# Autodesk Inventor assembly: robot_frame_layer1
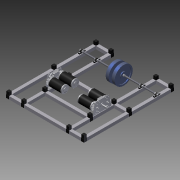
[picture p0: Inventor's stored thumbnail of the model, 180x180]
Saved by Autodesk Inventor 2011 (Build 150239000, 239)
## iProperties
Created: 2013-01-17
Part Number: robot_frame_layer1
Document SubType Name: Assembly
Designer: Christopher
Author: Christopher
## Documents named in this file (19)
- F:\Users\Christopher\Documents\GitHub\2013CAD\2013 robot\forklift\robot parts\robot_frame_layer1.iam
- F:\Users\Christopher\Documents\GitHub\2013CAD\2013 robot\forklift\robot parts\1tube_4_layer1_outside.ipt
- F:\Users\Christopher\Documents\GitHub\2013CAD\2013 robot\forklift\robot parts\1tube_6_layer1_boardsupportsupport.ipt
- F:\Users\Christopher\Documents\GitHub\2013CAD\2013 robot\forklift\robot parts\1tube_6_layer1_motorsupport.ipt
- F:\Users\Christopher\Documents\GitHub\2013CAD\2013 robot\forklift\robot parts\1tube_14_layer1_innersupport.ipt
- F:\Users\Christopher\Documents\GitHub\2013CAD\2013 robot\forklift\robot parts\1tube_14_layer1_inside.ipt
- F:\Users\Christopher\Documents\GitHub\2013CAD\2013 robot\forklift\robot parts\1tube_14_layer1_outside.ipt
- F:\Users\Christopher\Documents\GitHub\2013CAD\2013 robot\forklift\Misc parts\3-way corner.ipt
- F:\Users\Christopher\Documents\GitHub\2013CAD\2013 robot\forklift\Misc parts\4-way corner.ipt
- F:\Users\Christopher\Documents\GitHub\2013CAD\2013 robot\forklift\Misc parts\5-way corner.ipt
- F:\Users\Christopher\Documents\GitHub\2013CAD\2013 robot\forklift\robot parts\1tube_13_layer1_side.ipt
- F:\Users\Christopher\Documents\GitHub\2013CAD\2013 robot\forklift\Chassis\Chassis_CIMGearbox_AndyMark_am-0734.ipt
- F:\Users\Christopher\Documents\GitHub\2013CAD\2013 robot\forklift\Misc parts\.5inch_side_bearing.ipt
- F:\Users\Christopher\Documents\GitHub\2013CAD\2013 robot\forklift\Misc parts\1.5_bolt_.25_20.ipt
- F:\Users\Christopher\Documents\GitHub\2013CAD\2013 robot\forklift\Misc parts\nut_.25_20.ipt
- F:\Users\Christopher\Documents\GitHub\2013CAD\2013 robot\forklift\Misc parts\.5_inch_axle_bushing.ipt
- F:\Users\Christopher\Documents\GitHub\2013CAD\2013 robot\forklift\robot parts\example_wheel_6inch_.5axle.ipt
- F:\Users\Christopher\Documents\GitHub\2013CAD\2013 robot\forklift\frame parts\0.5unkeyedaxle_26.ipt
- F:\Users\Christopher\Documents\GitHub\2013CAD\2013 robot\forklift\frame parts\corner_prop.ipt
## Components (70 placed, 18 different names)
1. 1tube_4_layer1_outside:1 — Mate:7, Mate:8, Mate:9, Mate:10, Mate:11, Mate:12
2. 1tube_6_layer1_boardsupportsupport:1 — Mate:22, Mate:23, Mate:24, Mate:25, Mate:26, Mate:27
3. 1tube_6_layer1_motorsupport:1 — Mate:28, Mate:29, Mate:30, Mate:110, Flush:1, Mate:120, Flush:2
4. 1tube_14_layer1_innersupport:1 — Mate:31, Mate:32, Mate:33, Mate:46, Mate:47, Mate:48
5. 1tube_14_layer1_outside:1 — Mate:19, Mate:20, Mate:21, Mate:49, Mate:50, Mate:51
6. 3-way corner:1 — Mate:13, Mate:14, Mate:15, Mate:150, Mate:151
7. 3-way corner:2 — Mate:7, Mate:8, Mate:9, Mate:148
8. 3-way corner:4 — Mate:70, Mate:71, Mate:72, Mate:121, Mate:122, Mate:131
9. 3-way corner:5 — Mate:73, Mate:74, Mate:75, Mate:152, Flush:12, Flush:13, Mate:153
10. 3-way corner:6 — Mate:67, Mate:68, Mate:69, Flush:8, Flush:9
11. 3-way corner:7 — Mate:16, Mate:17, Mate:18, Mate:142, Mate:143, Mate:144
12. 4-way corner:2 — Mate:10, Mate:11, Mate:12, Mate:19, Mate:20, Mate:21, Mate:22, Mate:23, Mate:24
13. 1tube_4_layer1_outside:2 — Mate:13, Mate:14, Mate:15, Mate:16, Mate:17, Mate:18
14. 4-way corner:3 — Mate:25, Mate:26, Mate:27, Mate:28, Mate:29, Mate:30, Mate:31, Mate:32, Mate:33
15. 1tube_14_layer1_innersupport:2 — Mate:82, Mate:83, Mate:91, Mate:101, Mate:102, Mate:103
16. 4-way corner:5 — Mate:46, Mate:47, Mate:48, Mate:53, Mate:54, Mate:128, Mate:129, Mate:130
17. 4-way corner:6 — Mate:49, Mate:50, Mate:51, Mate:52, Mate:64, Mate:65, Mate:66
18. 1tube_6_layer1_motorsupport:2 — Mate:127, Flush:4, Flush:5, Mate:128, Mate:129, Mate:130, Mate:135, Mate:136, Mate:137
19. 1tube_6_layer1_boardsupportsupport:2 — Mate:52, Mate:53, Mate:54
20. 1tube_4_layer1_outside:3 — Mate:64, Mate:65, Mate:66, Mate:67, Mate:68, Mate:69
21. 1tube_4_layer1_outside:4 — Mate:70, Mate:71, Mate:72, Mate:73, Mate:74, Mate:75
22. 5-way corner:1 — Mate:82, Mate:83, Mate:85, Mate:86, Mate:87, Mate:91, Mate:123, Mate:124, Mate:125, Mate:126, Mate:135, Mate:136, Mate:137
23. 5-way corner:2 — Mate:101, Mate:102, Mate:103, Mate:110, Mate:116, Mate:139, Mate:140, Mate:141, Mate:147
24. 1tube_4_layer1_outside:5 — Mate:85, Mate:86, Mate:87, Mate:88, Mate:89, Mate:90
25. 4-way corner:7 — Mate:88, Mate:89, Mate:90, Mate:138, Flush:6, Flush:7
26. 4-way corner:8 — Mate:114, Mate:115, Mate:145, Flush:10, Flush:11, Mate:146, Mate:149
27. 1tube_4_layer1_outside:6 — Mate:114, Mate:115, Mate:116, Mate:146, Mate:147
28. Chassis_CIMGearbox_AndyMark_am-0734:1 — Flush:1, Mate:120, Flush:2
29. Chassis_CIMGearbox_AndyMark_am-0734:2 — Mate:127, Flush:4, Flush:5
30. 1tube_13_layer1_side:3 — Mate:121, Mate:122, Mate:123, Mate:124, Mate:125, Mate:126, Mate:131, Insert:1, Insert:2, Insert:11, Insert:12
31. 1tube_13_layer1_side:4 — Mate:152, Flush:12, Flush:13, Mate:153, Insert:25, Insert:26, Insert:31, Insert:32
32. 1tube_14_layer1_inside:2 — Mate:138, Flush:6, Flush:7, Flush:8, Flush:9
33. 1tube_14_layer1_inside:3 — Mate:145, Flush:10, Flush:11, Mate:148
34. 1tube_13_layer1_side:5 — Mate:139, Mate:140, Mate:141, Mate:142, Mate:143, Mate:144, Insert:3, Insert:4, Insert:9, Insert:10
35. 1tube_13_layer1_side:6 — Mate:149, Mate:150, Mate:151, Insert:23, Insert:24, Insert:33, Insert:34
36. .5inch_side_bearing:1 — Insert:1, Insert:2, Insert:5, Insert:6, Insert:18, Insert:35
37. .5inch_side_bearing:2 — Insert:3, Insert:4, Insert:7, Insert:8, Insert:19, Insert:36
38. 1.5_bolt_.25_20:1 — Insert:6
39. nut_.25_20:1 — Insert:9
40. 1.5_bolt_.25_20:2 — Insert:5
41. nut_.25_20:2 — Insert:10
42. 1.5_bolt_.25_20:3 — Insert:7
43. nut_.25_20:3 — Insert:12
44. 1.5_bolt_.25_20:4 — Insert:8
45. nut_.25_20:4 — Insert:11
46. .5_inch_axle_bushing:1 — Insert:16, Insert:18
47. .5_inch_axle_bushing:2 — Insert:17, Insert:19
48. example_wheel_6inch_.5axle:1 — Insert:16, Insert:20
49. example_wheel_6inch_.5axle:2 — Insert:17, Insert:21, Insert:22
50. .5_inch_axle_bushing:3 — Insert:22
51. .5_inch_axle_bushing:4 — Insert:21
52. .5_inch_axle_bushing:5 — Insert:20
53. .5_inch_axle_bushing:6 — Insert:35
54. .5inch_side_bearing:3 — Insert:25, Insert:26, Insert:27, Insert:28, Insert:37, Insert:39
55. .5inch_side_bearing:4 — Insert:23, Insert:24, Insert:29, Insert:30, Insert:38, Insert:40
56. 1.5_bolt_.25_20:5 — Insert:28
57. 1.5_bolt_.25_20:6 — Insert:30
58. 1.5_bolt_.25_20:7 — Insert:29
59. 1.5_bolt_.25_20:8 — Insert:27
60. nut_.25_20:5 — Insert:32
61. nut_.25_20:6 — Insert:31
62. nut_.25_20:7 — Insert:34
63. nut_.25_20:8 — Insert:33
64. .5_inch_axle_bushing:7 — Insert:36
65. .5_inch_axle_bushing:8 — Insert:37, Insert:41
66. .5_inch_axle_bushing:9 — Insert:38
67. .5_inch_axle_bushing:10 — Insert:39
68. .5_inch_axle_bushing:11 — Insert:40
69. 0.5unkeyedaxle_26:1 — Insert:41
70. corner_prop:1
## Relationships (145: Mate 95, Insert 38, Flush 12)
- Mate:7: 1tube_4_layer1_outside:1 ↔ 3-way corner:2
- Mate:8: 1tube_4_layer1_outside:1 ↔ 3-way corner:2
- Mate:9: 1tube_4_layer1_outside:1 ↔ 3-way corner:2
- Mate:10: 1tube_4_layer1_outside:1 ↔ 4-way corner:2
- Mate:11: 1tube_4_layer1_outside:1 ↔ 4-way corner:2
- Mate:12: 1tube_4_layer1_outside:1 ↔ 4-way corner:2
- Mate:13: 3-way corner:1 ↔ 1tube_4_layer1_outside:2
- Mate:14: 3-way corner:1 ↔ 1tube_4_layer1_outside:2
- Mate:15: 3-way corner:1 ↔ 1tube_4_layer1_outside:2
- Mate:16: 3-way corner:7 ↔ 1tube_4_layer1_outside:2
- Mate:17: 3-way corner:7 ↔ 1tube_4_layer1_outside:2
- Mate:18: 3-way corner:7 ↔ 1tube_4_layer1_outside:2
- Mate:19: 1tube_14_layer1_outside:1 ↔ 4-way corner:2
- Mate:20: 1tube_14_layer1_outside:1 ↔ 4-way corner:2
- Mate:21: 1tube_14_layer1_outside:1 ↔ 4-way corner:2
- Mate:22: 1tube_6_layer1_boardsupportsupport:1 ↔ 4-way corner:2
- Mate:23: 1tube_6_layer1_boardsupportsupport:1 ↔ 4-way corner:2
- Mate:24: 1tube_6_layer1_boardsupportsupport:1 ↔ 4-way corner:2
- Mate:25: 1tube_6_layer1_boardsupportsupport:1 ↔ 4-way corner:3
- Mate:26: 1tube_6_layer1_boardsupportsupport:1 ↔ 4-way corner:3
- Mate:27: 1tube_6_layer1_boardsupportsupport:1 ↔ 4-way corner:3
- Mate:28: 1tube_6_layer1_motorsupport:1 ↔ 4-way corner:3
- Mate:29: 1tube_6_layer1_motorsupport:1 ↔ 4-way corner:3
- Mate:30: 1tube_6_layer1_motorsupport:1 ↔ 4-way corner:3
- Mate:31: 1tube_14_layer1_innersupport:1 ↔ 4-way corner:3
- Mate:32: 1tube_14_layer1_innersupport:1 ↔ 4-way corner:3
- Mate:33: 1tube_14_layer1_innersupport:1 ↔ 4-way corner:3
- Mate:46: 1tube_14_layer1_innersupport:1 ↔ 4-way corner:5
- Mate:47: 1tube_14_layer1_innersupport:1 ↔ 4-way corner:5
- Mate:48: 1tube_14_layer1_innersupport:1 ↔ 4-way corner:5
- Mate:49: 1tube_14_layer1_outside:1 ↔ 4-way corner:6
- Mate:50: 1tube_14_layer1_outside:1 ↔ 4-way corner:6
- Mate:51: 1tube_14_layer1_outside:1 ↔ 4-way corner:6
- Mate:52: 4-way corner:6 ↔ 1tube_6_layer1_boardsupportsupport:2
- Mate:53: 4-way corner:5 ↔ 1tube_6_layer1_boardsupportsupport:2
- Mate:54: 4-way corner:5 ↔ 1tube_6_layer1_boardsupportsupport:2
- Mate:64: 4-way corner:6 ↔ 1tube_4_layer1_outside:3
- Mate:65: 4-way corner:6 ↔ 1tube_4_layer1_outside:3
- Mate:66: 4-way corner:6 ↔ 1tube_4_layer1_outside:3
- Mate:67: 3-way corner:6 ↔ 1tube_4_layer1_outside:3
- Mate:68: 3-way corner:6 ↔ 1tube_4_layer1_outside:3
- Mate:69: 3-way corner:6 ↔ 1tube_4_layer1_outside:3
- Mate:70: 3-way corner:4 ↔ 1tube_4_layer1_outside:4
- Mate:71: 3-way corner:4 ↔ 1tube_4_layer1_outside:4
- Mate:72: 3-way corner:4 ↔ 1tube_4_layer1_outside:4
- Mate:73: 3-way corner:5 ↔ 1tube_4_layer1_outside:4
- Mate:74: 3-way corner:5 ↔ 1tube_4_layer1_outside:4
- Mate:75: 3-way corner:5 ↔ 1tube_4_layer1_outside:4
- Mate:82: 1tube_14_layer1_innersupport:2 ↔ 5-way corner:1
- Mate:83: 1tube_14_layer1_innersupport:2 ↔ 5-way corner:1
- Mate:85: 5-way corner:1 ↔ 1tube_4_layer1_outside:5
- Mate:86: 5-way corner:1 ↔ 1tube_4_layer1_outside:5
- Mate:87: 5-way corner:1 ↔ 1tube_4_layer1_outside:5
- Mate:88: 1tube_4_layer1_outside:5 ↔ 4-way corner:7
- Mate:89: 1tube_4_layer1_outside:5 ↔ 4-way corner:7
- Mate:90: 1tube_4_layer1_outside:5 ↔ 4-way corner:7
- Mate:91: 1tube_14_layer1_innersupport:2 ↔ 5-way corner:1
- Mate:101: 1tube_14_layer1_innersupport:2 ↔ 5-way corner:2
- Mate:102: 1tube_14_layer1_innersupport:2 ↔ 5-way corner:2
- Mate:103: 1tube_14_layer1_innersupport:2 ↔ 5-way corner:2
- Mate:110: 1tube_6_layer1_motorsupport:1 ↔ 5-way corner:2
- Mate:114: 4-way corner:8 ↔ 1tube_4_layer1_outside:6
- Mate:115: 4-way corner:8 ↔ 1tube_4_layer1_outside:6
- Mate:116: 5-way corner:2 ↔ 1tube_4_layer1_outside:6
- Flush:1: 1tube_6_layer1_motorsupport:1 ↔ Chassis_CIMGearbox_AndyMark_am-0734:1
- Mate:120: 1tube_6_layer1_motorsupport:1 ↔ Chassis_CIMGearbox_AndyMark_am-0734:1
- Mate:121: 3-way corner:4 ↔ 1tube_13_layer1_side:3
- Mate:122: 3-way corner:4 ↔ 1tube_13_layer1_side:3
- Mate:123: 5-way corner:1 ↔ 1tube_13_layer1_side:3
- Mate:124: 5-way corner:1 ↔ 1tube_13_layer1_side:3
- Mate:125: 5-way corner:1 ↔ 1tube_13_layer1_side:3
- Mate:126: 5-way corner:1 ↔ 1tube_13_layer1_side:3
- Flush:2: 1tube_6_layer1_motorsupport:1 ↔ Chassis_CIMGearbox_AndyMark_am-0734:1
- Mate:127: 1tube_6_layer1_motorsupport:2 ↔ Chassis_CIMGearbox_AndyMark_am-0734:2
- Flush:4: 1tube_6_layer1_motorsupport:2 ↔ Chassis_CIMGearbox_AndyMark_am-0734:2
- Flush:5: 1tube_6_layer1_motorsupport:2 ↔ Chassis_CIMGearbox_AndyMark_am-0734:2
- Mate:128: 4-way corner:5 ↔ 1tube_6_layer1_motorsupport:2
- Mate:129: 4-way corner:5 ↔ 1tube_6_layer1_motorsupport:2
- Mate:130: 4-way corner:5 ↔ 1tube_6_layer1_motorsupport:2
- Mate:131: 3-way corner:4 ↔ 1tube_13_layer1_side:3
- Mate:135: 1tube_6_layer1_motorsupport:2 ↔ 5-way corner:1
- Mate:136: 1tube_6_layer1_motorsupport:2 ↔ 5-way corner:1
- Mate:137: 1tube_6_layer1_motorsupport:2 ↔ 5-way corner:1
- Mate:138: 4-way corner:7 ↔ 1tube_14_layer1_inside:2
- Flush:6: 4-way corner:7 ↔ 1tube_14_layer1_inside:2
- Flush:7: 4-way corner:7 ↔ 1tube_14_layer1_inside:2
- Flush:8: 3-way corner:6 ↔ 1tube_14_layer1_inside:2
- Flush:9: 3-way corner:6 ↔ 1tube_14_layer1_inside:2
- Mate:139: 5-way corner:2 ↔ 1tube_13_layer1_side:5
- Mate:140: 5-way corner:2 ↔ 1tube_13_layer1_side:5
- Mate:141: 5-way corner:2 ↔ 1tube_13_layer1_side:5
- Mate:142: 3-way corner:7 ↔ 1tube_13_layer1_side:5
- Mate:143: 3-way corner:7 ↔ 1tube_13_layer1_side:5
- Mate:144: 3-way corner:7 ↔ 1tube_13_layer1_side:5
- Mate:145: 4-way corner:8 ↔ 1tube_14_layer1_inside:3
- Flush:10: 4-way corner:8 ↔ 1tube_14_layer1_inside:3
- Flush:11: 4-way corner:8 ↔ 1tube_14_layer1_inside:3
- Mate:146: 4-way corner:8 ↔ 1tube_4_layer1_outside:6
- Mate:147: 5-way corner:2 ↔ 1tube_4_layer1_outside:6
- Mate:148: 3-way corner:2 ↔ 1tube_14_layer1_inside:3
- Mate:149: 4-way corner:8 ↔ 1tube_13_layer1_side:6
- Mate:150: 3-way corner:1 ↔ 1tube_13_layer1_side:6
- Mate:151: 3-way corner:1 ↔ 1tube_13_layer1_side:6
- Mate:152: 3-way corner:5 ↔ 1tube_13_layer1_side:4
- Flush:12: 3-way corner:5 ↔ 1tube_13_layer1_side:4
- Flush:13: 3-way corner:5 ↔ 1tube_13_layer1_side:4
- Mate:153: 3-way corner:5 ↔ 1tube_13_layer1_side:4
- Insert:1: 1tube_13_layer1_side:3 ↔ .5inch_side_bearing:1
- Insert:2: 1tube_13_layer1_side:3 ↔ .5inch_side_bearing:1
- Insert:3: 1tube_13_layer1_side:5 ↔ .5inch_side_bearing:2
- Insert:4: 1tube_13_layer1_side:5 ↔ .5inch_side_bearing:2
- Insert:5: .5inch_side_bearing:1 ↔ 1.5_bolt_.25_20:2
- Insert:6: .5inch_side_bearing:1 ↔ 1.5_bolt_.25_20:1
- Insert:7: .5inch_side_bearing:2 ↔ 1.5_bolt_.25_20:3
- Insert:8: .5inch_side_bearing:2 ↔ 1.5_bolt_.25_20:4
- Insert:9: 1tube_13_layer1_side:5 ↔ nut_.25_20:1
- Insert:10: 1tube_13_layer1_side:5 ↔ nut_.25_20:2
- Insert:11: 1tube_13_layer1_side:3 ↔ nut_.25_20:4
- Insert:12: 1tube_13_layer1_side:3 ↔ nut_.25_20:3
- Insert:16 (165.1 mm): .5_inch_axle_bushing:1 ↔ example_wheel_6inch_.5axle:1
- Insert:17 (165.1 mm): .5_inch_axle_bushing:2 ↔ example_wheel_6inch_.5axle:2
- Insert:18: .5inch_side_bearing:1 ↔ .5_inch_axle_bushing:1
- Insert:19: .5inch_side_bearing:2 ↔ .5_inch_axle_bushing:2
- Insert:20: example_wheel_6inch_.5axle:1 ↔ .5_inch_axle_bushing:5
- Insert:21: example_wheel_6inch_.5axle:2 ↔ .5_inch_axle_bushing:4
- Insert:22: example_wheel_6inch_.5axle:2 ↔ .5_inch_axle_bushing:3
- Insert:23: 1tube_13_layer1_side:6 ↔ .5inch_side_bearing:4
- Insert:24: 1tube_13_layer1_side:6 ↔ .5inch_side_bearing:4
- Insert:25: 1tube_13_layer1_side:4 ↔ .5inch_side_bearing:3
- Insert:26: 1tube_13_layer1_side:4 ↔ .5inch_side_bearing:3
- Insert:27: .5inch_side_bearing:3 ↔ 1.5_bolt_.25_20:8
- Insert:28: .5inch_side_bearing:3 ↔ 1.5_bolt_.25_20:5
- Insert:29: .5inch_side_bearing:4 ↔ 1.5_bolt_.25_20:7
- Insert:30: .5inch_side_bearing:4 ↔ 1.5_bolt_.25_20:6
- Insert:31: 1tube_13_layer1_side:4 ↔ nut_.25_20:6
- Insert:32: 1tube_13_layer1_side:4 ↔ nut_.25_20:5
- Insert:33: 1tube_13_layer1_side:6 ↔ nut_.25_20:8
- Insert:34: 1tube_13_layer1_side:6 ↔ nut_.25_20:7
- Insert:35: .5inch_side_bearing:1 ↔ .5_inch_axle_bushing:6
- Insert:36: .5inch_side_bearing:2 ↔ .5_inch_axle_bushing:7
- Insert:37: .5inch_side_bearing:3 ↔ .5_inch_axle_bushing:8
- Insert:38: .5inch_side_bearing:4 ↔ .5_inch_axle_bushing:9
- Insert:39: .5inch_side_bearing:3 ↔ .5_inch_axle_bushing:10
- Insert:40: .5inch_side_bearing:4 ↔ .5_inch_axle_bushing:11
- Insert:41: .5_inch_axle_bushing:8 ↔ 0.5unkeyedaxle_26:1
